# Autodesk Inventor assembly: WBR
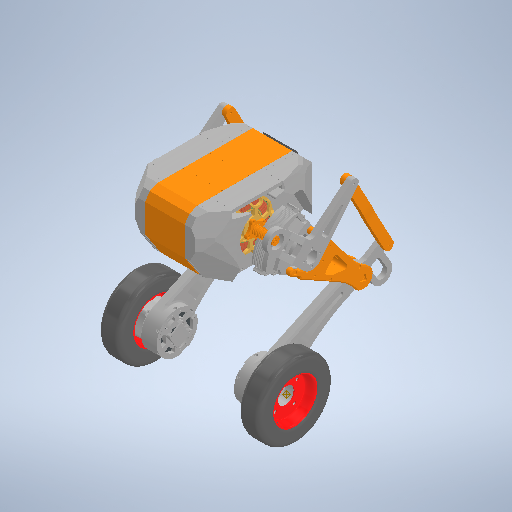
[picture p0: Inventor's stored thumbnail of the model, 512x512]
Saved by Autodesk Inventor 2025.2 (Build 292293000, 293)
## iProperties
Created: 2025-04-16
Part Number: WBR
Document SubType Name: Assembly
Designer: Bruno
Author: Bruno
## Documents named in this file (32)
- D:\Universidad\Ciclo 9\PROYECTO INTEGRADOR III\BIPEDO\WBR\WBR.iam
- D:\Universidad\Ciclo 9\PROYECTO INTEGRADOR III\BIPEDO\Pierna V1\Llanta Bipedo.ipt
- D:\Universidad\Ciclo 9\PROYECTO INTEGRADOR III\BIPEDO\WBR\Pierna_L V2\BLDC_GIM6010_reductor.ipt
- D:\Universidad\Ciclo 9\PROYECTO INTEGRADOR III\BIPEDO\WBR\Pierna_L V2\acople_llanta.ipt
- D:\Universidad\Ciclo 9\PROYECTO INTEGRADOR III\BIPEDO\WBR\Pierna_L V2\BLDC_GIM6010.ipt
- D:\Universidad\Ciclo 9\PROYECTO INTEGRADOR III\BIPEDO\WBR\Pierna_L V2\leg_wheel.ipt
- D:\Universidad\Ciclo 9\PROYECTO INTEGRADOR III\BIPEDO\WBR\Pierna_L V2\oDrive_micro_housing.ipt
- D:\Universidad\Ciclo 9\PROYECTO INTEGRADOR III\BIPEDO\WBR\Pierna_L V2\leg_extend.ipt
- D:\Universidad\Ciclo 9\PROYECTO INTEGRADOR III\BIPEDO\WBR\Pierna_L V2\motion_thigh_bot.ipt
- D:\Universidad\Ciclo 9\PROYECTO INTEGRADOR III\BIPEDO\WBR\Pierna_L V2\motion_thigh_top.ipt
- D:\Universidad\Ciclo 9\PROYECTO INTEGRADOR III\BIPEDO\WBR\Pierna_L V2\thigh_joint.ipt
- D:\Universidad\Ciclo 9\PROYECTO INTEGRADOR III\BIPEDO\WBR\Pierna_L V2\driven_thigh.ipt
- D:\Universidad\Ciclo 9\PROYECTO INTEGRADOR III\BIPEDO\WBR\Pierna_L V2\REDUCTOR CAPSTAN\Big_drum.ipt
- D:\Universidad\Ciclo 9\PROYECTO INTEGRADOR III\BIPEDO\WBR\Pierna_L V2\REDUCTOR CAPSTAN\Brace.ipt
- D:\Universidad\Ciclo 9\PROYECTO INTEGRADOR III\BIPEDO\WBR\Pierna_L V2\REDUCTOR CAPSTAN\Small_drum.ipt
- D:\Universidad\Ciclo 9\PROYECTO INTEGRADOR III\BIPEDO\WBR\Pierna_L V2\Eagle_Power_8308_BLDC\Rotor.ipt
- D:\Universidad\Ciclo 9\PROYECTO INTEGRADOR III\BIPEDO\WBR\Pierna_L V2\Eagle_Power_8308_BLDC\Stator.ipt
- D:\Universidad\Ciclo 9\PROYECTO INTEGRADOR III\BIPEDO\WBR\Pierna_L V2\body_side.ipt
- D:\Universidad\Ciclo 9\PROYECTO INTEGRADOR III\BIPEDO\WBR\Pierna_R V2\leg_wheel_R.ipt
- D:\Universidad\Ciclo 9\PROYECTO INTEGRADOR III\BIPEDO\WBR\Pierna_R V2\motion_thigh_bot_R.ipt
- D:\Universidad\Ciclo 9\PROYECTO INTEGRADOR III\BIPEDO\WBR\Pierna_R V2\motion_thigh_top_R.ipt
- D:\Universidad\Ciclo 9\PROYECTO INTEGRADOR III\BIPEDO\WBR\Pierna_R V2\REDUCTOR CAPSTAN\Big_drum_R.ipt
- D:\Universidad\Ciclo 9\PROYECTO INTEGRADOR III\BIPEDO\WBR\Pierna_R V2\REDUCTOR CAPSTAN\Brace_R.ipt
- D:\Universidad\Ciclo 9\PROYECTO INTEGRADOR III\BIPEDO\WBR\Pierna_R V2\REDUCTOR CAPSTAN\Small_drum_R.ipt
- D:\Universidad\Ciclo 9\PROYECTO INTEGRADOR III\BIPEDO\WBR\OUT_SHELL.ipt
- D:\Universidad\Ciclo 9\PROYECTO INTEGRADOR III\BIPEDO\WBR\Pierna_R V2\body_side_R2.ipt
- D:\Universidad\Ciclo 9\PROYECTO INTEGRADOR III\BIPEDO\WBR\OUT_SHELL_R.ipt
- D:\Universidad\Ciclo 9\PROYECTO INTEGRADOR III\BIPEDO\WBR\inner_body_b.ipt
- D:\Universidad\Ciclo 9\PROYECTO INTEGRADOR III\BIPEDO\WBR\inner_body_c.ipt
- D:\Universidad\Ciclo 9\PROYECTO INTEGRADOR III\BIPEDO\WBR\Pierna_R V2\leg_extend_R.ipt
- D:\Universidad\Ciclo 9\PROYECTO INTEGRADOR III\BIPEDO\WBR\Voltimetro Amperimetro 0 -100 V 0 - 10 A.ipt
- D:\Universidad\Ciclo 9\PROYECTO INTEGRADOR III\BIPEDO\WBR\Pierna_L V2\oDrive_micro_cover.ipt
## Components (41 placed, 30 different names)
1. acople_llanta:1 — Mate:3, Mate:4, Mate:5, Mate:10, Mate:132, Mate:133, Mate:148
2. Llanta Bipedo:1 — Tangent:2, Mate:1, Mate:2, Mate:3, Mate:4, Mate:5, Mate:41, Angle:40, Mate:59, Flush:13, Symmetry:4
3. Llanta Bipedo:2 — Angle:40, Flush:3, Tangent:3, Mate:59, Mate:60, Mate:61, Mate:62, Flush:14, Symmetry:5
4. acople_llanta:2 — Mate:60, Mate:61, Mate:62, Mate:67, Mate:134, Mate:135
5. oDrive_micro_cover:2 — Mate:161, Mate:162, Mate:163
6. leg_wheel:1 — Mate:11, Mate:12, Mate:13, Mate:14, Mate:15, Mate:16, Mate:17, Mate:18, Mate:19
7. oDrive_micro_housing:1 — Mate:15, Mate:16, Mate:161, Mate:162, Mate:163
8. leg_extend:1 — Mate:17, Mate:18, Mate:19, Mate:20, Flush:2, Mate:27, Mate:28, Mate:39, Mate:48
9. motion_thigh_bot:1 — Mate:21, Mate:22, Mate:23
10. motion_thigh_top:1 — Mate:29, Mate:30, Mate:31, Mate:40, Mate:46, Mate:47, Mate:48, Mate:146
11. thigh_joint:1 — Mate:20, Flush:2, Mate:21, Mate:22, Mate:23, Mate:46, Mate:47
12. driven_thigh:1 — Mate:27, Mate:28, Mate:33, Mate:34, Mate:43
13. Rotor:1 — Mate:49, Mate:50, Mate:51
14. Stator:1 — Mate:56, Mate:57, Mate:58
15. Big_drum:1 — JOINT ANGLE, Mate:29, Mate:30, Mate:31, Mate:32, Mate:44, Rotation:1, Angle:42, REORDENAR
16. Brace:1 — Mate:32, Mate:33, Mate:34, Mate:35, Mate:36, Angle:37, Mate:42, Mate:53, Mate:54, Mate:55, Angle:41, Mate:145
17. Small_drum_body:1 — Mate:35, Mate:36, Rotation:1, Mate:49, Mate:50, Mate:51, REORDENAR
18. Voltimetro Amperimetro 0 -100 V 0 - 10 A:1 — Mate:164, Mate:165, Mate:166
19. body_side:1 — Mate:53, Mate:54, Mate:55, Mate:56, Mate:57, Mate:58, Mate:119, Mate:120, Mate:121, Mate:131, Flush:11, Flush:12, Mate:140, Symmetry:1
20. body_side_r:1 — Mate:122, Mate:123, Mate:124, Mate:125, Mate:126, Mate:127, Mate:128, Mate:129, Flush:6, Mate:130, Flush:7, Flush:9, Flush:10
21. OUT_SHELL:1 — Mate:119, Mate:120, Mate:121, Symmetry:2
22. OUT_SHELL_R:1 — Mate:127, Mate:128, Mate:129, Symmetry:2
23. inner_body_b:1 — Flush:6, Mate:130, Flush:7, Mate:140, Symmetry:3
24. inner_body_c:1 — Flush:9, Flush:10, Mate:131, Flush:11, Flush:12, Symmetry:1, Symmetry:3, Mate:164, Mate:165, Mate:166
25. Rotor:2 — Mate:99, Mate:100
26. Big_drum_R:1 — Mate:90, Mate:91, Mate:92, Mate:93, Angle:42, Rotation:2, Mate:141
27. Brace_R:1 — Mate:88, Mate:89, Mate:90, Angle:41, Mate:94, Mate:95, Mate:124, Mate:125, Mate:126, Mate:141
28. Small_drum_body_R:1 — Mate:94, Mate:95, Rotation:2, Mate:99, Mate:100
29. Stator:2 — Mate:122, Mate:123
30. oDrive_micro_cover:1 — Mate:158, Mate:159, Mate:160
31. leg_extend:2 — Mate:136, Mate:137, Mate:139
32. leg_wheel_R:1 — Mate:68, Mate:69, Mate:70, Flush:4, Mate:71, Mate:72, Mate:136, Mate:138
33. oDrive_micro_housing:2 — Flush:4, Mate:71, Mate:72, Mate:158, Mate:159, Mate:160
34. motion_thigh_top_R:1 — Mate:80, Mate:81, Mate:82, Mate:91, Mate:153
35. motion_thigh_bot_R:1 — Mate:77, Mate:78, Mate:79, Mate:92, Mate:93
36. driven_thigh:2 — Mate:88, Mate:89, Mate:137
37. thigh_joint:2 — Mate:77, Mate:78, Mate:79, Mate:80, Mate:81, Mate:82, Mate:138, Mate:139
38. BLDC_GIM6010:1 — Mate:6, Mate:7, Mate:11, Mate:12, Mate:13, Mate:14
39. BLDC_GIM6010_reductor:1 — Mate:6, Mate:7, Mate:10, Mate:132, Mate:133
40. BLDC_GIM6010_reductor:2 — Mate:67, Mate:134, Mate:135
41. BLDC_GIM6010:2 — Mate:68, Mate:69, Mate:70
## Relationships (151: Mate 123, Flush 13, Angle 6, Symmetry 5, Tangent 2, RelateRotation 2)
- Flush:1 (-73.05 mm)
- Tangent:2: Llanta Bipedo:1
- Mate:1: Llanta Bipedo:1
- Mate:2 (116 mm): Llanta Bipedo:1
- Mate:3: acople_llanta:1 ↔ Llanta Bipedo:1
- Mate:4: acople_llanta:1 ↔ Llanta Bipedo:1
- Mate:5: acople_llanta:1 ↔ Llanta Bipedo:1
- Mate:6: BLDC_GIM6010:1 ↔ BLDC_GIM6010_reductor:1
- Mate:7: BLDC_GIM6010:1 ↔ BLDC_GIM6010_reductor:1
- Mate:10: acople_llanta:1 ↔ BLDC_GIM6010_reductor:1
- Mate:11: leg_wheel:1 ↔ BLDC_GIM6010:1
- Mate:12: leg_wheel:1 ↔ BLDC_GIM6010:1
- Mate:13: leg_wheel:1 ↔ BLDC_GIM6010:1
- Mate:14: leg_wheel:1 ↔ BLDC_GIM6010:1
- Mate:15: leg_wheel:1 ↔ oDrive_micro_housing:1
- Mate:16: leg_wheel:1 ↔ oDrive_micro_housing:1
- Mate:17: leg_wheel:1 ↔ leg_extend:1
- Mate:18: leg_wheel:1 ↔ leg_extend:1
- Mate:19: leg_wheel:1 ↔ leg_extend:1
- Mate:20: leg_extend:1 ↔ thigh_joint:1
- Flush:2: leg_extend:1 ↔ thigh_joint:1
- Mate:21: motion_thigh_bot:1 ↔ thigh_joint:1
- Mate:22: motion_thigh_bot:1 ↔ thigh_joint:1
- Mate:23: motion_thigh_bot:1 ↔ thigh_joint:1
- Mate:27: leg_extend:1 ↔ driven_thigh:1
- Mate:28: leg_extend:1 ↔ driven_thigh:1
- JOINT ANGLE [Angle] (-41 deg): Big_drum:1
- Mate:29: motion_thigh_top:1 ↔ Big_drum:1
- Mate:30: motion_thigh_top:1 ↔ Big_drum:1
- Mate:31: motion_thigh_top:1 ↔ Big_drum:1
- Mate:32: Big_drum:1 ↔ Brace:1
- Mate:33: driven_thigh:1 ↔ Brace:1
- Mate:34: driven_thigh:1 ↔ Brace:1
- Mate:35: Brace:1 ↔ Small_drum_body:1
- Mate:36: Brace:1 ↔ Small_drum_body:1
- Angle:37 (-131 deg): Brace:1
- Angle:39 (0 deg)
- Mate:39: leg_extend:1
- Mate:40: motion_thigh_top:1
- Mate:41: Llanta Bipedo:1
- Mate:42: Brace:1
- Mate:43: driven_thigh:1
- Mate:44: Big_drum:1
- Mate:45
- Mate:46: motion_thigh_top:1 ↔ thigh_joint:1
- Mate:47: motion_thigh_top:1 ↔ thigh_joint:1
- Mate:48: leg_extend:1 ↔ motion_thigh_top:1
- Rotation:1 [RelateRotation] (0.125 ul): Big_drum:1 ↔ Small_drum_body:1
- Mate:49: Rotor:1 ↔ Small_drum_body:1
- Mate:50: Rotor:1 ↔ Small_drum_body:1
- Mate:51: Rotor:1 ↔ Small_drum_body:1
- Mate:53: Brace:1 ↔ body_side:1
- Mate:54: Brace:1 ↔ body_side:1
- Mate:55: Brace:1 ↔ body_side:1
- Mate:56: Stator:1 ↔ body_side:1
- Mate:57: Stator:1 ↔ body_side:1
- Mate:58: Stator:1 ↔ body_side:1
- Angle:40 (0 deg): Llanta Bipedo:1 ↔ Llanta Bipedo:2
- Flush:3 (116 mm): Llanta Bipedo:2
- Tangent:3: Llanta Bipedo:2
- Mate:59: Llanta Bipedo:1 ↔ Llanta Bipedo:2
- Mate:60: Llanta Bipedo:2 ↔ acople_llanta:2
- Mate:61: Llanta Bipedo:2 ↔ acople_llanta:2
- Mate:62: Llanta Bipedo:2 ↔ acople_llanta:2
- [Mate]: BLDC_GIM6010_reductor:2 ↔ BLDC_GIM6010:2
- [Mate]: BLDC_GIM6010_reductor:2 ↔ BLDC_GIM6010:2
- Mate:67: acople_llanta:2 ↔ BLDC_GIM6010_reductor:2
- Mate:68: leg_wheel_R:1 ↔ BLDC_GIM6010:2
- Mate:69: leg_wheel_R:1 ↔ BLDC_GIM6010:2
- Mate:70: leg_wheel_R:1 ↔ BLDC_GIM6010:2
- Flush:4: leg_wheel_R:1 ↔ oDrive_micro_housing:2
- Mate:71: leg_wheel_R:1 ↔ oDrive_micro_housing:2
- Mate:72: leg_wheel_R:1 ↔ oDrive_micro_housing:2
- Mate:77: motion_thigh_bot_R:1 ↔ thigh_joint:2
- Mate:78: motion_thigh_bot_R:1 ↔ thigh_joint:2
- Mate:79: motion_thigh_bot_R:1 ↔ thigh_joint:2
- Mate:80: motion_thigh_top_R:1 ↔ thigh_joint:2
- Mate:81: motion_thigh_top_R:1 ↔ thigh_joint:2
- Mate:82: motion_thigh_top_R:1 ↔ thigh_joint:2
- Mate:88: Brace_R:1 ↔ driven_thigh:2
- Mate:89: Brace_R:1 ↔ driven_thigh:2
- Mate:90: Big_drum_R:1 ↔ Brace_R:1
- Mate:91: Big_drum_R:1 ↔ motion_thigh_top_R:1
- Mate:92: Big_drum_R:1 ↔ motion_thigh_bot_R:1
- Mate:93: Big_drum_R:1 ↔ motion_thigh_bot_R:1
- Angle:41 (0 deg): Brace:1 ↔ Brace_R:1
- Angle:42 (0 deg): Big_drum:1 ↔ Big_drum_R:1
- Mate:94: Brace_R:1 ↔ Small_drum_body_R:1
- Mate:95: Brace_R:1 ↔ Small_drum_body_R:1
- Rotation:2 [RelateRotation] (0.125 ul): Big_drum_R:1 ↔ Small_drum_body_R:1
- Mate:99: Rotor:2 ↔ Small_drum_body_R:1
- Mate:100: Rotor:2 ↔ Small_drum_body_R:1
- Mate:119: body_side:1 ↔ OUT_SHELL:1
- Mate:120: body_side:1 ↔ OUT_SHELL:1
- Mate:121: body_side:1 ↔ OUT_SHELL:1
- Mate:122: body_side_r:1 ↔ Stator:2
- Mate:123: body_side_r:1 ↔ Stator:2
- Mate:124: body_side_r:1 ↔ Brace_R:1
- Mate:125: body_side_r:1 ↔ Brace_R:1
- Mate:126: body_side_r:1 ↔ Brace_R:1
- Mate:127: body_side_r:1 ↔ OUT_SHELL_R:1
- Mate:128: body_side_r:1 ↔ OUT_SHELL_R:1
- Mate:129: body_side_r:1 ↔ OUT_SHELL_R:1
- Flush:6: body_side_r:1 ↔ inner_body_b:1
- Mate:130: body_side_r:1 ↔ inner_body_b:1
- Flush:7: body_side_r:1 ↔ inner_body_b:1
- REORDENAR [Flush]: Big_drum:1 ↔ Small_drum_body:1
- Flush:9: body_side_r:1 ↔ inner_body_c:1
- Flush:10: body_side_r:1 ↔ inner_body_c:1
- Mate:131: body_side:1 ↔ inner_body_c:1
- Mate:132: acople_llanta:1 ↔ BLDC_GIM6010_reductor:1
- Mate:133: acople_llanta:1 ↔ BLDC_GIM6010_reductor:1
- Mate:134: acople_llanta:2 ↔ BLDC_GIM6010_reductor:2
- Mate:135: acople_llanta:2 ↔ BLDC_GIM6010_reductor:2
- Mate:136: leg_extend:2 ↔ leg_wheel_R:1
- Mate:137: leg_extend:2 ↔ driven_thigh:2
- Mate:138: leg_wheel_R:1 ↔ thigh_joint:2
- Mate:139: leg_extend:2 ↔ thigh_joint:2
- Flush:11: body_side:1 ↔ inner_body_c:1
- Flush:12: body_side:1 ↔ inner_body_c:1
- Mate:140: body_side:1 ↔ inner_body_b:1
- Mate:141: Big_drum_R:1 ↔ Brace_R:1
- Symmetry:1: body_side:1 ↔ inner_body_c:1
- Symmetry:2: OUT_SHELL:1 ↔ OUT_SHELL_R:1
- Symmetry:3: inner_body_b:1 ↔ inner_body_c:1
- Mate:142
- Mate:143
- Mate:144
- Mate:145: Brace:1
- Mate:146: motion_thigh_top:1
- Mate:147
- Mate:148: acople_llanta:1
- Flush:13: Llanta Bipedo:1
- Symmetry:4: Llanta Bipedo:1
- Flush:14: Llanta Bipedo:2
- Symmetry:5: Llanta Bipedo:2
- Mate:149
- Mate:150
- Mate:151
- Mate:152
- Mate:153: motion_thigh_top_R:1
- Mate:154
- Mate:158: oDrive_micro_cover:1 ↔ oDrive_micro_housing:2
- Mate:159: oDrive_micro_cover:1 ↔ oDrive_micro_housing:2
- Mate:160: oDrive_micro_cover:1 ↔ oDrive_micro_housing:2
- Mate:161: oDrive_micro_cover:2 ↔ oDrive_micro_housing:1
- Mate:162: oDrive_micro_cover:2 ↔ oDrive_micro_housing:1
- Mate:163: oDrive_micro_cover:2 ↔ oDrive_micro_housing:1
- Mate:164: Voltimetro Amperimetro 0 -100 V 0 - 10 A:1 ↔ inner_body_c:1
- Mate:165: Voltimetro Amperimetro 0 -100 V 0 - 10 A:1 ↔ inner_body_c:1
- Mate:166: Voltimetro Amperimetro 0 -100 V 0 - 10 A:1 ↔ inner_body_c:1
## Named parameters: d91_d11 = 0 mm, d92_d12 = 0 mm, Finish10_Area = 892.124, Finish10_Thickness = 0 mm, Finish11_Area = 916.245, Finish11_Thickness = 0 mm, Finish12_Area = 98.7132, Finish12_Thickness = 0 mm, Finish13_Area = 55.4009, Finish13_Thickness = 0 mm, Finish14_Area = 55.4009, Finish14_Thickness = 0 mm, Finish1_Area = 124.027, Finish1_Thickness = 0.05 mm, Finish2_Area = 9.72009, Finish2_Thickness = 0.05 mm, Finish3_Area = 124.027, Finish3_Thickness = 0.05 mm, Finish4_Area = 1359.48, Finish4_Thickness = 0 mm, Finish5_Area = 1110, Finish5_Thickness = 0 mm, Finish6_Area = 3286.79, Finish6_Thickness = 0 mm, Finish7_Area = 458.122, Finish7_Thickness = 0 mm, Finish8_Area = 1683.29, Finish8_Thickness = 0 mm, Finish9_Area = 892.124, Finish9_Thickness = 0 mm
note: some values were not read from the file. Shown as the stored number, unit unknown: "Finish10_Area", "Finish11_Area", "Finish12_Area", "Finish13_Area", "Finish14_Area", "Finish1_Area", "Finish2_Area", "Finish3_Area", "Finish4_Area", "Finish5_Area", "Finish6_Area", "Finish7_Area", "Finish8_Area", "Finish9_Area".
